# Autodesk Inventor assembly: Pelvis
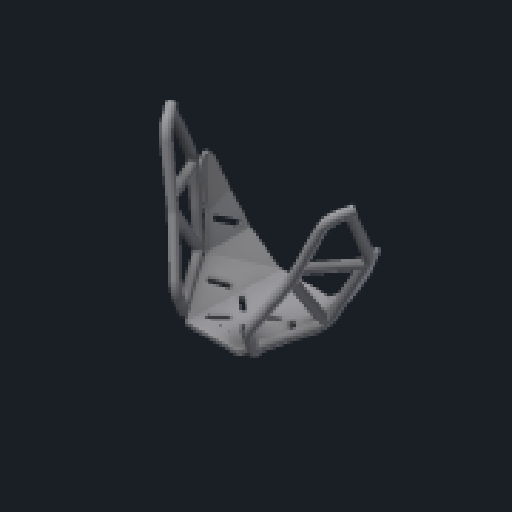
[picture p0: Inventor's stored thumbnail of the model, 512x512]
Saved by Autodesk Inventor 2025.2 (Build 292293000, 293)
## iProperties
Created: 2020-05-05
Part Number: Pelvis
Document SubType Name: Assembly
Designer: valer
Author: valer
## Documents named in this file (3)
- C:\Users\valer\Desktop\str1ker\cad\Pelvis.iam
- C:\Users\valer\Desktop\str1ker\cad\SpineLinkRoot.ipt
- C:\Users\valer\Desktop\str1ker\cad\PelvisWing.ipt
## Components (3 placed, 2 different names)
1. SpineLinkRoot:1 — Mate:1, Mate:2
2. PelvisWing:3
3. PelvisWing:4
## Relationships (2: Mate 2)
- Mate:1: SpineLinkRoot:1
- Mate:2: SpineLinkRoot:1
